# Autodesk Inventor assembly: Support A Assembly
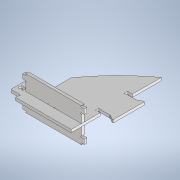
[picture p0: Inventor's stored thumbnail of the model, 180x180]
Saved by Autodesk Inventor 2020 (Build 240168000, 168)
## iProperties
Created: 2020-05-11
Part Number: Support A Assembly
Document SubType Name: Assembly
Designer: Dan Wikman
Author: Dan Wikman
## Documents named in this file (3)
- C:\Users\Dan Wikman\OneDrive\University Life\2020, Semester 1\METR4900 Honours Thesis\Full Scale Design\Support A Assembly.iam
- C:\Users\Dan Wikman\OneDrive\University Life\2020, Semester 1\METR4900 Honours Thesis\Full Scale Design\Layer 1 Plank.ipt
- C:\Users\Dan Wikman\OneDrive\University Life\2020, Semester 1\METR4900 Honours Thesis\Full Scale Design\Support A.ipt
## Components (3 placed, 2 different names)
1. Layer 1 Plank:1 — Mate:3, Flush:2, Mate:4
2. Layer 1 Plank:4 — Mate:1, Mate:2, Flush:1
3. Support A:1 — Mate:1, Mate:2, Flush:1, Mate:3, Flush:2, Mate:4
## Relationships (6: Mate 4, Flush 2)
- Mate:1: Layer 1 Plank:4 ↔ Support A:1
- Mate:2 (0.5 mm): Layer 1 Plank:4 ↔ Support A:1
- Flush:1: Layer 1 Plank:4 ↔ Support A:1
- Mate:3: Layer 1 Plank:1 ↔ Support A:1
- Flush:2: Layer 1 Plank:1 ↔ Support A:1
- Mate:4 (0.5 mm): Layer 1 Plank:1 ↔ Support A:1
